# Autodesk Inventor assembly: LI0003-CASE ASSY
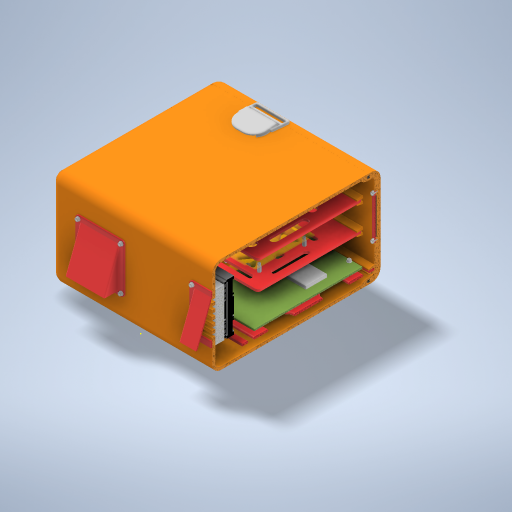
[picture p0: Inventor's stored thumbnail of the model, 512x512]
Saved by Autodesk Inventor 2023 (Build 270158000, 158)
## iProperties
Created: 2023-03-14
Part Number: LI0003-CASE ASSY
Document SubType Name: Assembly
Designer: Louis
Mass: 1323.99 g
Surface Area: 3900.17 cm^2
Volume: 1323.99 cm^3
Density: 1 g/cm^3
Author: Louis
## Documents named in this file (15)
- D:\Louis\Documents\Inventor\Interferometry\LIA0003-CASE ASSY.iam
- D:\Louis\Documents\Inventor\Interferometry\LI0001-CASE BODY.ipt
- D:\Louis\Documents\Inventor\Interferometry\LI0005-SEAL.ipt
- D:\Louis\Documents\Inventor\Interferometry\LI0006-CLASP.ipt
- D:\Louis\Documents\Inventor\Interferometry\LI0007-LATCH.ipt
- D:\Louis\Documents\Inventor\Interferometry\FAN SPACE MODEL.ipt
- D:\Louis\Documents\Inventor\Interferometry\LIA0002-LID ASSY.iam
- D:\Louis\Documents\Inventor\Interferometry\rcp-080-t_3D.iam
- D:\Louis\Documents\Inventor\Interferometry\LI0010-FAN SHROUD.ipt
- D:\Louis\Documents\Inventor\Interferometry\LI0013-FOOT.ipt
- D:\Louis\Documents\Inventor\Interferometry\LATCH TEST MP.ipt
- D:\Louis\Documents\Inventor\Interferometry\LI0008-LATCH PIN.ipt
- D:\Louis\Documents\Inventor\Interferometry\M3 WASHER.ipt
- D:\Louis\Documents\Inventor\Interferometry\M3 X 10.ipt
- D:\Louis\Documents\Inventor\Interferometry\M3 X 25.ipt
## Components (76 placed, 14 different names)
1. LI0001-CASE BODY:1 — Mate:10, Mate:11, Mate:12, Mate:15, Mate:16, Mate:17, Mate:18, Mate:19, Mate:20, Mate:21, Mate:22, Mate:23, Mate:24, Mate:25, Mate:26, Mate:31, Mate:32, Mate:33, Mate:34, Mate:35, Mate:36, Mate:39, Mate:40, Mate:41, Mate:42, Mate:43, Mate:44, Mate:45, Mate:46, Mate:47, Mate:48, Mate:49, Mate:50, Mate:53, Mate:54, Mate:55, Mate:56, Mate:57, Mate:58, Mate:59, Mate:60, Mate:61, Mate:62, Mate:63, Mate:64, Mate:65, Mate:66, Mate:67, Mate:68, Mate:69, Mate:70, Mate:71, Mate:72, Mate:73, Mate:74, Mate:75, Mate:76, Angle:1, Angle:2, Angle:3, Angle:4, Angle:5, Angle:6, Angle:7, Angle:8, Mate:77, Insert:17, Insert:18, Insert:19, Insert:20
2. LI0005-SEAL:1 — Mate:21, Mate:22, Mate:23
3. FAN SPACE MODEL:1 — Mate:15, Mate:16, Mate:17, Mate:27, Flush:1, Flush:2
4. LIA0002-LID ASSY:1 [sub-assembly] — Mate:18, Mate:19, Mate:20
5. FAN SPACE MODEL:2 — Mate:24, Mate:25, Mate:26, Mate:28, Flush:3, Flush:4
6. rcp-080-t_3D:1 [sub-assembly] — Mate:27, Flush:1, Flush:2
7. rcp-080-t_3D:2 [sub-assembly] — Mate:28, Flush:3, Flush:4
8. FAN SPACE MODEL:3 — Mate:31, Mate:32, Mate:33, Mate:38, Flush:7, Flush:8
9. FAN SPACE MODEL:4 — Mate:34, Mate:35, Mate:36, Mate:37, Flush:5, Flush:6
10. rcp-080-t_3D:3 [sub-assembly] — Mate:37, Flush:5, Flush:6
11. rcp-080-t_3D:4 [sub-assembly] — Mate:38, Flush:7, Flush:8
12. LI0010-FAN SHROUD:1 — Mate:39, Mate:40, Mate:41, Insert:25, Insert:26, Insert:27, Insert:28
13. LI0010-FAN SHROUD:2 — Mate:45, Mate:46, Mate:47, Insert:33, Insert:34, Insert:35, Insert:36
14. LI0010-FAN SHROUD:3 — Mate:42, Mate:43, Mate:44, Insert:21, Insert:22, Insert:23, Insert:24
15. LI0010-FAN SHROUD:4 — Mate:48, Mate:49, Mate:50, Insert:37, Insert:38, Insert:39, Insert:40
16. LI0006-CLASP:2 — Insert:7, Insert:8, Angle:6, Insert:13
17. LI0006-CLASP:3 — Insert:3, Insert:10, Angle:3, Insert:16
18. LI0006-CLASP:4 — Insert:6, Insert:9, Angle:5, Insert:14
19. LI0007-LATCH:2 — Insert:7, Angle:7
20. LI0007-LATCH:3 — Insert:3, Angle:4
21. LI0007-LATCH:4 — Insert:6, Angle:8
22. LI0013-FOOT:1 — Mate:56, Mate:57, Mate:58
23. LI0013-FOOT:2 — Mate:59, Mate:60, Mate:61
24. LI0013-FOOT:3 — Mate:53, Mate:54, Mate:55
25. LI0013-FOOT:4 — Mate:62, Mate:63, Mate:64
26. LATCH TEST MP:1 — Mate:71, Mate:72, Mate:73, Insert:8
27. LATCH TEST MP:2 — Mate:65, Mate:66, Mate:67, Insert:10
28. LATCH TEST MP:3 — Mate:68, Mate:69, Mate:70, Insert:11
29. LATCH TEST MP:4 — Mate:74, Mate:75, Mate:76, Insert:9
30. LI0006-CLASP:5 — Insert:11, Insert:12, Angle:1, Insert:15
31. LI0007-LATCH:5 — Insert:12, Angle:2
32. LI0008-LATCH PIN:1 — Insert:16
33. LI0008-LATCH PIN:2 — Insert:15
34. LI0008-LATCH PIN:3 — Insert:14
35. LI0008-LATCH PIN:4 — Insert:13
36. LI0010-FAN SHROUD:5 — Mate:77, Insert:17, Insert:18, Insert:19, Insert:20, Insert:29, Insert:30, Insert:31, Insert:32
37. M3 WASHER:1 — Insert:31, Insert:59
38. M3 WASHER:2 — Insert:29, Insert:58
39. M3 WASHER:3 — Insert:32, Insert:60
40. M3 WASHER:4 — Insert:30, Insert:57
41. M3 WASHER:5 — Insert:26, Insert:41
42. M3 WASHER:6 — Insert:25, Insert:43
43. M3 WASHER:7 — Insert:27, Insert:42
44. M3 WASHER:8 — Insert:28, Insert:44
45. M3 WASHER:9 — Insert:24, Insert:48
46. M3 WASHER:10 — Insert:23, Insert:46
47. M3 WASHER:11 — Insert:21, Insert:45
48. M3 WASHER:12 — Insert:22, Insert:47
49. M3 WASHER:13 — Insert:36, Insert:51
50. M3 WASHER:14 — Insert:33, Insert:52
51. M3 WASHER:15 — Insert:35, Insert:50
52. M3 WASHER:16 — Insert:34, Insert:49
53. M3 WASHER:17 — Insert:37, Insert:53
54. M3 WASHER:18 — Insert:40, Insert:56
55. M3 WASHER:19 — Insert:38, Insert:54
56. M3 WASHER:20 — Insert:39, Insert:55
57. M3 X 25:1 — Insert:49
58. M3 X 25:2 — Insert:56
59. M3 X 25:3 — Insert:50
60. M3 X 25:4 — Insert:55
61. M3 X 25:5 — Insert:51
62. M3 X 25:6 — Insert:52
63. M3 X 25:7 — Insert:53
64. M3 X 25:8 — Insert:54
65. M3 X 25:9 — Insert:46
66. M3 X 25:10 — Insert:45
67. M3 X 25:11 — Insert:47
68. M3 X 25:12 — Insert:48
69. M3 X 25:13 — Insert:41
70. M3 X 25:14 — Insert:43
71. M3 X 25:15 — Insert:42
72. M3 X 25:16 — Insert:44
73. M3 X 10:1 — Insert:57
74. M3 X 10:2 — Insert:59
75. M3 X 10:3 — Insert:58
76. M3 X 10:4 — Insert:60
## Relationships (134: Mate 62, Insert 56, Flush 8, Angle 8)
- Mate:10: LI0001-CASE BODY:1
- Mate:11: LI0001-CASE BODY:1
- Mate:12: LI0001-CASE BODY:1
- Mate:15: LI0001-CASE BODY:1 ↔ FAN SPACE MODEL:1
- Mate:16: LI0001-CASE BODY:1 ↔ FAN SPACE MODEL:1
- Mate:17: LI0001-CASE BODY:1 ↔ FAN SPACE MODEL:1
- Mate:18: LI0001-CASE BODY:1 ↔ LIA0002-LID ASSY:1
- Mate:19: LI0001-CASE BODY:1 ↔ LIA0002-LID ASSY:1
- Mate:20: LI0001-CASE BODY:1 ↔ LIA0002-LID ASSY:1
- Mate:21: LI0001-CASE BODY:1 ↔ LI0005-SEAL:1
- Mate:22: LI0001-CASE BODY:1 ↔ LI0005-SEAL:1
- Mate:23: LI0001-CASE BODY:1 ↔ LI0005-SEAL:1
- Mate:24: LI0001-CASE BODY:1 ↔ FAN SPACE MODEL:2
- Mate:25: LI0001-CASE BODY:1 ↔ FAN SPACE MODEL:2
- Mate:26: LI0001-CASE BODY:1 ↔ FAN SPACE MODEL:2
- Mate:27: FAN SPACE MODEL:1 ↔ rcp-080-t_3D:1
- Flush:1: FAN SPACE MODEL:1 ↔ rcp-080-t_3D:1
- Flush:2: FAN SPACE MODEL:1 ↔ rcp-080-t_3D:1
- Mate:28: FAN SPACE MODEL:2 ↔ rcp-080-t_3D:2
- Flush:3: FAN SPACE MODEL:2 ↔ rcp-080-t_3D:2
- Flush:4: FAN SPACE MODEL:2 ↔ rcp-080-t_3D:2
- Mate:31: LI0001-CASE BODY:1 ↔ FAN SPACE MODEL:3
- Mate:32: LI0001-CASE BODY:1 ↔ FAN SPACE MODEL:3
- Mate:33: LI0001-CASE BODY:1 ↔ FAN SPACE MODEL:3
- Mate:34: LI0001-CASE BODY:1 ↔ FAN SPACE MODEL:4
- Mate:35: LI0001-CASE BODY:1 ↔ FAN SPACE MODEL:4
- Mate:36: LI0001-CASE BODY:1 ↔ FAN SPACE MODEL:4
- Mate:37: FAN SPACE MODEL:4 ↔ rcp-080-t_3D:3
- Flush:5: FAN SPACE MODEL:4 ↔ rcp-080-t_3D:3
- Flush:6: FAN SPACE MODEL:4 ↔ rcp-080-t_3D:3
- Mate:38: FAN SPACE MODEL:3 ↔ rcp-080-t_3D:4
- Flush:7: FAN SPACE MODEL:3 ↔ rcp-080-t_3D:4
- Flush:8: FAN SPACE MODEL:3 ↔ rcp-080-t_3D:4
- Mate:39: LI0001-CASE BODY:1 ↔ LI0010-FAN SHROUD:1
- Mate:40: LI0001-CASE BODY:1 ↔ LI0010-FAN SHROUD:1
- Mate:41: LI0001-CASE BODY:1 ↔ LI0010-FAN SHROUD:1
- Mate:42: LI0001-CASE BODY:1 ↔ LI0010-FAN SHROUD:3
- Mate:43: LI0001-CASE BODY:1 ↔ LI0010-FAN SHROUD:3
- Mate:44: LI0001-CASE BODY:1 ↔ LI0010-FAN SHROUD:3
- Mate:45: LI0001-CASE BODY:1 ↔ LI0010-FAN SHROUD:2
- Mate:46: LI0001-CASE BODY:1 ↔ LI0010-FAN SHROUD:2
- Mate:47: LI0001-CASE BODY:1 ↔ LI0010-FAN SHROUD:2
- Mate:48: LI0001-CASE BODY:1 ↔ LI0010-FAN SHROUD:4
- Mate:49: LI0001-CASE BODY:1 ↔ LI0010-FAN SHROUD:4
- Mate:50: LI0001-CASE BODY:1 ↔ LI0010-FAN SHROUD:4
- Insert:3: LI0006-CLASP:3 ↔ LI0007-LATCH:3
- Insert:6: LI0006-CLASP:4 ↔ LI0007-LATCH:4
- Insert:7: LI0006-CLASP:2 ↔ LI0007-LATCH:2
- Mate:53: LI0001-CASE BODY:1 ↔ LI0013-FOOT:3
- Mate:54: LI0001-CASE BODY:1 ↔ LI0013-FOOT:3
- Mate:55: LI0001-CASE BODY:1 ↔ LI0013-FOOT:3
- Mate:56: LI0001-CASE BODY:1 ↔ LI0013-FOOT:1
- Mate:57: LI0001-CASE BODY:1 ↔ LI0013-FOOT:1
- Mate:58: LI0001-CASE BODY:1 ↔ LI0013-FOOT:1
- Mate:59: LI0001-CASE BODY:1 ↔ LI0013-FOOT:2
- Mate:60: LI0001-CASE BODY:1 ↔ LI0013-FOOT:2
- Mate:61: LI0001-CASE BODY:1 ↔ LI0013-FOOT:2
- Mate:62: LI0001-CASE BODY:1 ↔ LI0013-FOOT:4
- Mate:63: LI0001-CASE BODY:1 ↔ LI0013-FOOT:4
- Mate:64: LI0001-CASE BODY:1 ↔ LI0013-FOOT:4
- Mate:65: LI0001-CASE BODY:1 ↔ LATCH TEST MP:2
- Mate:66: LI0001-CASE BODY:1 ↔ LATCH TEST MP:2
- Mate:67: LI0001-CASE BODY:1 ↔ LATCH TEST MP:2
- Mate:68: LI0001-CASE BODY:1 ↔ LATCH TEST MP:3
- Mate:69: LI0001-CASE BODY:1 ↔ LATCH TEST MP:3
- Mate:70: LI0001-CASE BODY:1 ↔ LATCH TEST MP:3
- Mate:71: LI0001-CASE BODY:1 ↔ LATCH TEST MP:1
- Mate:72: LI0001-CASE BODY:1 ↔ LATCH TEST MP:1
- Mate:73: LI0001-CASE BODY:1 ↔ LATCH TEST MP:1
- Mate:74: LI0001-CASE BODY:1 ↔ LATCH TEST MP:4
- Mate:75: LI0001-CASE BODY:1 ↔ LATCH TEST MP:4
- Mate:76: LI0001-CASE BODY:1 ↔ LATCH TEST MP:4
- Insert:8: LI0006-CLASP:2 ↔ LATCH TEST MP:1
- Insert:9: LI0006-CLASP:4 ↔ LATCH TEST MP:4
- Insert:10: LI0006-CLASP:3 ↔ LATCH TEST MP:2
- Insert:11: LATCH TEST MP:3 ↔ LI0006-CLASP:5
- Insert:12: LI0006-CLASP:5 ↔ LI0007-LATCH:5
- Angle:1 (180 deg): LI0001-CASE BODY:1 ↔ LI0006-CLASP:5
- Angle:2 (185 deg): LI0001-CASE BODY:1 ↔ LI0007-LATCH:5
- Angle:3 (180 deg): LI0001-CASE BODY:1 ↔ LI0006-CLASP:3
- Angle:4 (185 deg): LI0001-CASE BODY:1 ↔ LI0007-LATCH:3
- Angle:5 (180 deg): LI0001-CASE BODY:1 ↔ LI0006-CLASP:4
- Angle:6 (180 deg): LI0001-CASE BODY:1 ↔ LI0006-CLASP:2
- Angle:7 (175 deg): LI0001-CASE BODY:1 ↔ LI0007-LATCH:2
- Angle:8 (175 deg): LI0001-CASE BODY:1 ↔ LI0007-LATCH:4
- Insert:13: LI0006-CLASP:2 ↔ LI0008-LATCH PIN:4
- Insert:14: LI0006-CLASP:4 ↔ LI0008-LATCH PIN:3
- Insert:15: LI0006-CLASP:5 ↔ LI0008-LATCH PIN:2
- Insert:16: LI0006-CLASP:3 ↔ LI0008-LATCH PIN:1
- Mate:77: LI0001-CASE BODY:1 ↔ LI0010-FAN SHROUD:5
- Insert:17: LI0001-CASE BODY:1 ↔ LI0010-FAN SHROUD:5
- Insert:18: LI0001-CASE BODY:1 ↔ LI0010-FAN SHROUD:5
- Insert:19: LI0001-CASE BODY:1 ↔ LI0010-FAN SHROUD:5
- Insert:20: LI0001-CASE BODY:1 ↔ LI0010-FAN SHROUD:5
- Insert:21: LI0010-FAN SHROUD:3 ↔ M3 WASHER:11
- Insert:22: LI0010-FAN SHROUD:3 ↔ M3 WASHER:12
- Insert:23: LI0010-FAN SHROUD:3 ↔ M3 WASHER:10
- Insert:24: LI0010-FAN SHROUD:3 ↔ M3 WASHER:9
- Insert:25: LI0010-FAN SHROUD:1 ↔ M3 WASHER:6
- Insert:26: LI0010-FAN SHROUD:1 ↔ M3 WASHER:5
- Insert:27: LI0010-FAN SHROUD:1 ↔ M3 WASHER:7
- Insert:28: LI0010-FAN SHROUD:1 ↔ M3 WASHER:8
- Insert:29: LI0010-FAN SHROUD:5 ↔ M3 WASHER:2
- Insert:30: LI0010-FAN SHROUD:5 ↔ M3 WASHER:4
- Insert:31: LI0010-FAN SHROUD:5 ↔ M3 WASHER:1
- Insert:32: LI0010-FAN SHROUD:5 ↔ M3 WASHER:3
- Insert:33: LI0010-FAN SHROUD:2 ↔ M3 WASHER:14
- Insert:34: LI0010-FAN SHROUD:2 ↔ M3 WASHER:16
- Insert:35: LI0010-FAN SHROUD:2 ↔ M3 WASHER:15
- Insert:36: LI0010-FAN SHROUD:2 ↔ M3 WASHER:13
- Insert:37: LI0010-FAN SHROUD:4 ↔ M3 WASHER:17
- Insert:38: LI0010-FAN SHROUD:4 ↔ M3 WASHER:19
- Insert:39: LI0010-FAN SHROUD:4 ↔ M3 WASHER:20
- Insert:40: LI0010-FAN SHROUD:4 ↔ M3 WASHER:18
- Insert:41: M3 WASHER:5 ↔ M3 X 25:13
- Insert:42: M3 WASHER:7 ↔ M3 X 25:15
- Insert:43: M3 WASHER:6 ↔ M3 X 25:14
- Insert:44: M3 WASHER:8 ↔ M3 X 25:16
- Insert:45: M3 WASHER:11 ↔ M3 X 25:10
- Insert:46: M3 WASHER:10 ↔ M3 X 25:9
- Insert:47: M3 WASHER:12 ↔ M3 X 25:11
- Insert:48: M3 WASHER:9 ↔ M3 X 25:12
- Insert:49: M3 WASHER:16 ↔ M3 X 25:1
- Insert:50: M3 WASHER:15 ↔ M3 X 25:3
- Insert:51: M3 WASHER:13 ↔ M3 X 25:5
- Insert:52: M3 WASHER:14 ↔ M3 X 25:6
- Insert:53: M3 WASHER:17 ↔ M3 X 25:7
- Insert:54: M3 WASHER:19 ↔ M3 X 25:8
- Insert:55: M3 WASHER:20 ↔ M3 X 25:4
- Insert:56: M3 WASHER:18 ↔ M3 X 25:2
- Insert:57: M3 WASHER:4 ↔ M3 X 10:1
- Insert:58: M3 WASHER:2 ↔ M3 X 10:3
- Insert:59: M3 WASHER:1 ↔ M3 X 10:2
- Insert:60: M3 WASHER:3 ↔ M3 X 10:4
